# Autodesk Inventor assembly: 下半身
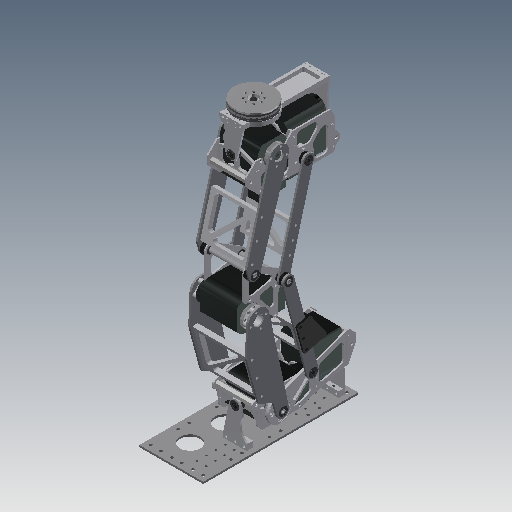
[picture p0: Inventor's stored thumbnail of the model, 512x512]
Saved by Autodesk Inventor 2017.3 (Build 213256000, 256)
## iProperties
Created: 2016-04-27
Part Number: 下半身
Document SubType Name: Assembly
Designer: hiroaki
Mass: 907.113 g
Surface Area: 2198.73 cm^2
Volume: 403.531 cm^3
Density: 2.24794 g/cm^3
Author: hiroaki
## Documents named in this file (11)
- C:\Users\haya\Desktop\GankenKun0_5\下半身_MIR.iam
- C:\Users\haya\Desktop\GankenKun0_5\下半身\リンク\ふともも\リンク_ふともも_前_1.iam
- C:\Users\haya\Desktop\GankenKun0_5\下半身\リンク\ふくらはぎ\リンク_ふくらはぎ_前_1.iam
- C:\Users\haya\Desktop\GankenKun0_5\下半身\リンク\ふくらはぎ\リンク_ふくらはぎ_後ろ_1.iam
- C:\Users\haya\Desktop\GankenKun0_5\下半身\付け根ロール\付け根ロール_1_MIR.iam
- C:\Users\haya\Desktop\GankenKun0_5\下半身\付け根\付け根_1_MIR.iam
- C:\Users\haya\Desktop\GankenKun0_5\下半身\膝\膝_1_1_MIR.iam
- C:\Users\haya\Desktop\GankenKun0_5\下半身\リンク\ふともも\リンク_ふともも_後ろ_1_MIR.iam
- C:\Users\haya\Desktop\GankenKun0_5\下半身\足裏\足裏_1_1_MIR.iam
- C:\Users\haya\Desktop\GankenKun0_5\下半身\足首\足首_1_MIR.iam
- C:\Users\haya\Desktop\GankenKun0_5\下半身\足首\足首_独立ピッチ_1.iam
## Components (10 placed, 10 different names)
1. 付け根ロール_1_MIR:1 [sub-assembly] — 角度:20, 挿入:25, 挿入:26, 角度:14, 角度:15, 角度:16, 角度:25
2. 付け根_1_MIR:1 [sub-assembly] — 挿入:25, 挿入:26, 挿入:27, 角度:14, 角度:15, 角度:16, 挿入:28, 挿入:31, 角度:25, 挿入:51
3. リンク_ふともも_前_1:1 [sub-assembly] — 挿入:27, 挿入:28, 挿入:30, 角度:18, 角度:19, 角度:26, 角度:22, 挿入:50, 角度:28
4. リンク_ふくらはぎ_前_1:1 [sub-assembly] — 角度:23, 角度:24, 挿入:46, 挿入:47, 挿入:48, 挿入:49, 角度:27, 角度:17, 角度:29
5. リンク_ふくらはぎ_後ろ_1:1 [sub-assembly] — 挿入:39, 挿入:40, 挿入:44, 挿入:45, 角度:29
6. 膝_1_1_MIR:1 [sub-assembly] — 挿入:30, 角度:17, 角度:22, 角度:18, 角度:24, 角度:19, 角度:23, 角度:26, 角度:27, 挿入:48, 挿入:49, 挿入:50, 挿入:52
7. リンク_ふともも_後ろ_1_MIR:1 [sub-assembly] — 挿入:31, 挿入:39, 挿入:40, 挿入:51, 挿入:52, 角度:28
8. 足裏_1_1_MIR:1 [sub-assembly] — 角度:20, 挿入:41, 挿入:42
9. 足首_1_MIR:1 [sub-assembly] — 挿入:41, 挿入:42, 挿入:43
10. 足首_独立ピッチ_1:1 [sub-assembly] — 挿入:43, 挿入:44, 挿入:45, 挿入:46, 挿入:47
## Relationships (35: Insert 20, Angle 15)
- 角度:20 [Angle] (0 deg): 付け根ロール_1_MIR:1 ↔ 足裏_1_1_MIR:1
- 挿入:25 [Insert]: 付け根ロール_1_MIR:1 ↔ 付け根_1_MIR:1
- 挿入:26 [Insert]: 付け根ロール_1_MIR:1 ↔ 付け根_1_MIR:1
- 挿入:27 [Insert]: 付け根_1_MIR:1 ↔ リンク_ふともも_前_1:1
- 角度:14 [Angle] (0 deg): 付け根ロール_1_MIR:1 ↔ 付け根_1_MIR:1
- 角度:15 [Angle] (45 deg): 付け根ロール_1_MIR:1 ↔ 付け根_1_MIR:1
- 角度:16 [Angle] (-20 deg): 付け根ロール_1_MIR:1 ↔ 付け根_1_MIR:1
- 挿入:28 [Insert]: 付け根_1_MIR:1 ↔ リンク_ふともも_前_1:1
- 挿入:30 [Insert]: リンク_ふともも_前_1:1 ↔ 膝_1_1_MIR:1
- 挿入:31 [Insert]: 付け根_1_MIR:1 ↔ リンク_ふともも_後ろ_1_MIR:1
- 角度:17 [Angle] (-15 deg): リンク_ふくらはぎ_前_1:1 ↔ 膝_1_1_MIR:1
- 角度:22 [Angle] (-15 deg): リンク_ふともも_前_1:1 ↔ 膝_1_1_MIR:1
- 角度:18 [Angle] (-80 deg): リンク_ふともも_前_1:1 ↔ 膝_1_1_MIR:1
- 角度:24 [Angle] (80 deg): リンク_ふくらはぎ_前_1:1 ↔ 膝_1_1_MIR:1
- 角度:19 [Angle] (-30 deg): リンク_ふともも_前_1:1 ↔ 膝_1_1_MIR:1
- 挿入:39 [Insert]: リンク_ふくらはぎ_後ろ_1:1 ↔ リンク_ふともも_後ろ_1_MIR:1
- 挿入:40 [Insert]: リンク_ふくらはぎ_後ろ_1:1 ↔ リンク_ふともも_後ろ_1_MIR:1
- 角度:23 [Angle] (-30 deg): リンク_ふくらはぎ_前_1:1 ↔ 膝_1_1_MIR:1
- 角度:25 [Angle] (20 deg): 付け根ロール_1_MIR:1 ↔ 付け根_1_MIR:1
- 挿入:41 [Insert]: 足裏_1_1_MIR:1 ↔ 足首_1_MIR:1
- 挿入:42 [Insert]: 足裏_1_1_MIR:1 ↔ 足首_1_MIR:1
- 挿入:43 [Insert]: 足首_1_MIR:1 ↔ 足首_独立ピッチ_1:1
- 挿入:44 [Insert]: リンク_ふくらはぎ_後ろ_1:1 ↔ 足首_独立ピッチ_1:1
- 挿入:45 [Insert]: リンク_ふくらはぎ_後ろ_1:1 ↔ 足首_独立ピッチ_1:1
- 挿入:46 [Insert]: リンク_ふくらはぎ_前_1:1 ↔ 足首_独立ピッチ_1:1
- 挿入:47 [Insert]: リンク_ふくらはぎ_前_1:1 ↔ 足首_独立ピッチ_1:1
- 角度:26 [Angle] (0 deg): リンク_ふともも_前_1:1 ↔ 膝_1_1_MIR:1
- 角度:27 [Angle] (0 deg): リンク_ふくらはぎ_前_1:1 ↔ 膝_1_1_MIR:1
- 挿入:48 [Insert]: リンク_ふくらはぎ_前_1:1 ↔ 膝_1_1_MIR:1
- 挿入:49 [Insert]: リンク_ふくらはぎ_前_1:1 ↔ 膝_1_1_MIR:1
- 挿入:50 [Insert]: リンク_ふともも_前_1:1 ↔ 膝_1_1_MIR:1
- 挿入:51 [Insert]: 付け根_1_MIR:1 ↔ リンク_ふともも_後ろ_1_MIR:1
- 挿入:52 [Insert]: 膝_1_1_MIR:1 ↔ リンク_ふともも_後ろ_1_MIR:1
- 角度:28 [Angle] (0 deg): リンク_ふともも_前_1:1 ↔ リンク_ふともも_後ろ_1_MIR:1
- 角度:29 [Angle] (0 deg): リンク_ふくらはぎ_前_1:1 ↔ リンク_ふくらはぎ_後ろ_1:1
